# Autodesk Inventor assembly: Assemlby_Scanner_v0
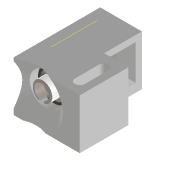
[picture p0: Inventor's stored thumbnail of the model, 180x180]
Saved by Autodesk Inventor 2022 (Build 260153000, 153)
## iProperties
Created: 2022-12-16
Part Number: Assemlby_Scanner_v0
Document SubType Name: Assembly
Designer: UC2
Author: UC2
## Documents named in this file (3)
- C:\Users\UC2\Documents\GitHub\Guinardia\INVENTOR\Assemlby_Scanner_v0.iam
- C:\Users\UC2\Documents\GitHub\Guinardia\INVENTOR\Assembly_Huawei_P30_Scanninglens.iam
- C:\Users\UC2\Documents\GitHub\Guinardia\INVENTOR\30_Scanlens_Laseradaper_v0.ipt
## Components (2 placed, 2 different names)
1. Assembly_Huawei_P30_Scanninglens:1 [sub-assembly] — Fluchtend:1, Fluchtend:2, Fluchtend:3
2. 30_Scanlens_Laseradaper_v0:1 — Fluchtend:1, Fluchtend:2, Fluchtend:3
## Relationships (3: Flush 3)
- Fluchtend:1 [Flush]: Assembly_Huawei_P30_Scanninglens:1 ↔ 30_Scanlens_Laseradaper_v0:1
- Fluchtend:2 [Flush]: Assembly_Huawei_P30_Scanninglens:1 ↔ 30_Scanlens_Laseradaper_v0:1
- Fluchtend:3 [Flush]: Assembly_Huawei_P30_Scanninglens:1 ↔ 30_Scanlens_Laseradaper_v0:1
